# Autodesk Inventor assembly: J005687
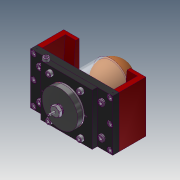
[picture p0: Inventor's stored thumbnail of the model, 180x180]
Saved by Autodesk Inventor 2015 SP1 (Build 190203100, 203)
## iProperties
Created: 2010-04-29
Part Number: J005687
Document SubType Name: Assembly
Designer: InventorUser
Description: CANNON AND HOLDER ASSY
Vendor: HHMI: JRC - ID&F
ALTERED ITEM DESCRIPTION: N/A
DESIGN DEPARTMENT: HHMI: JRC - ID&F
Revision Number: 0
## Documents named in this file (11)
- C:\_WORKSPACE\DATA\COLLABORATION\SVOBODA LAB\MOUSE POSITIONING SYSTEMS\MCAD\BALL SETUP\MBS AssemblyCanHolder.iam
- C:\_WORKSPACE\DATA\COLLABORATION\SVOBODA LAB\MOUSE POSITIONING SYSTEMS\MCAD\BALL SETUP\Ball_Rig\CanClamp.ipt
- C:\_WORKSPACE\DATA\COLLABORATION\SVOBODA LAB\MOUSE POSITIONING SYSTEMS\MCAD\BALL SETUP\Ball_Rig\CanClamper16.ipt
- C:\_WORKSPACE\DATA\COLLABORATION\SVOBODA LAB\MOUSE POSITIONING SYSTEMS\MCAD\BALL SETUP\Ball_Rig\ClamperPlate.ipt
- C:\_WORKSPACE\DATA\COLLABORATION\SVOBODA LAB\MOUSE POSITIONING SYSTEMS\MCAD\BALL SETUP\Ball_Rig\PingPongBall.ipt
- C:\_WORKSPACE\DATA\COLLABORATION\SVOBODA LAB\MOUSE POSITIONING SYSTEMS\MCAD\BALL SETUP\50745K150.ipt
- C:\_WORKSPACE\DATA\COLLABORATION\SVOBODA LAB\MOUSE POSITIONING SYSTEMS\MCAD\BALL SETUP\92185A203.ipt
- C:\_WORKSPACE\DATA\COLLABORATION\SVOBODA LAB\MOUSE POSITIONING SYSTEMS\MCAD\BALL SETUP\92185A194.ipt
- C:\_WORKSPACE\DATA\COLLABORATION\SVOBODA LAB\MOUSE POSITIONING SYSTEMS\MCAD\BALL SETUP\90291A578.ipt
- C:\_WORKSPACE\DATA\COLLABORATION\SVOBODA LAB\MOUSE POSITIONING SYSTEMS\MCAD\BALL SETUP\Ball_Rig\BottomCapAirBall.ipt
- C:\_WORKSPACE\DATA\COLLABORATION\SVOBODA LAB\MOUSE POSITIONING SYSTEMS\MCAD\BALL SETUP\Ball_Rig\BallHolderTubeAirBall.ipt
## Components (23 placed, 10 different names)
1. CanClamp:1 — Mate:1, Mate:2, Mate:7, Mate:8, Mate:12, Mate:13, Mate:34, Mate:35, Mate:36, Mate:37, Mate:38, Mate:39, Mate:40, Mate:41
2. CanClamper16:1 — Mate:3, Mate:4
3. CanClamper16:2 — Mate:5, Mate:6
4. ClamperPlate:1 — Mate:1, Mate:2, Mate:3, Mate:4, Mate:5, Mate:6, Mate:7, Mate:8, Mate:14, Mate:15, Mate:16, Mate:17, Mate:18, Mate:19, Mate:20, Mate:21, Mate:22, Mate:23, Mate:24, Mate:25, Mate:26, Mate:27, Flush:1, Mate:28, Flush:2, Mate:29, Flush:3, Mate:30, Flush:4
5. PingPongBall:1
6. 50745K150:1
7. 92185A203:1 — Mate:12, Mate:13
8. 92185A194:1 — Mate:14, Mate:15
9. 92185A194:2 — Mate:16, Mate:17
10. 92185A194:3 — Mate:18, Mate:19, Mate:20
11. 92185A194:4 — Mate:25, Mate:26
12. 92185A194:5 — Mate:23, Mate:24
13. 92185A194:6 — Mate:21, Mate:22
14. 90291A578:1 — Mate:28, Flush:2
15. 90291A578:2 — Mate:27, Flush:1
16. 90291A578:3 — Mate:29, Flush:3
17. 90291A578:4 — Mate:30, Flush:4
18. BottomCapAirBall:1
19. BallHolderTubeAirBall:1
20. 92185A194:7 — Mate:34, Mate:35
21. 92185A194:8 — Mate:36, Mate:37
22. 92185A194:9 — Mate:40, Mate:41
23. 92185A194:10 — Mate:38, Mate:39
## Relationships (46: Mate 41, Flush 4, Insert 1)
- Mate:1: CanClamp:1 ↔ ClamperPlate:1
- Mate:2: CanClamp:1 ↔ ClamperPlate:1
- Mate:3: CanClamper16:1 ↔ ClamperPlate:1
- Mate:4: CanClamper16:1 ↔ ClamperPlate:1
- Mate:5: CanClamper16:2 ↔ ClamperPlate:1
- Mate:6: CanClamper16:2 ↔ ClamperPlate:1
- Mate:7: CanClamp:1 ↔ ClamperPlate:1
- Mate:8: CanClamp:1 ↔ ClamperPlate:1
- [Insert] (-1.905 mm): CanClamp:1 ↔ BallHolderTubeAirBall:1
- [Mate]: PingPongBall:1 ↔ BallHolderTubeAirBall:1
- [Mate]: 50745K150:1 ↔ BottomCapAirBall:1
- [Mate] (2.54 mm): 50745K150:1 ↔ BottomCapAirBall:1
- Mate:12: CanClamp:1 ↔ 92185A203:1
- Mate:13: CanClamp:1 ↔ 92185A203:1
- Mate:14: ClamperPlate:1 ↔ 92185A194:1
- Mate:15: ClamperPlate:1 ↔ 92185A194:1
- Mate:16: ClamperPlate:1 ↔ 92185A194:2
- Mate:17: ClamperPlate:1 ↔ 92185A194:2
- Mate:18: ClamperPlate:1 ↔ 92185A194:3
- Mate:19: ClamperPlate:1 ↔ 92185A194:3
- Mate:20: ClamperPlate:1 ↔ 92185A194:3
- Mate:21: ClamperPlate:1 ↔ 92185A194:6
- Mate:22: ClamperPlate:1 ↔ 92185A194:6
- Mate:23: ClamperPlate:1 ↔ 92185A194:5
- Mate:24: ClamperPlate:1 ↔ 92185A194:5
- Mate:25: ClamperPlate:1 ↔ 92185A194:4
- Mate:26: ClamperPlate:1 ↔ 92185A194:4
- Mate:27: ClamperPlate:1 ↔ 90291A578:2
- Flush:1 (-2.54 mm): ClamperPlate:1 ↔ 90291A578:2
- Mate:28: ClamperPlate:1 ↔ 90291A578:1
- Flush:2 (-2.54 mm): ClamperPlate:1 ↔ 90291A578:1
- Mate:29: ClamperPlate:1 ↔ 90291A578:3
- Flush:3 (-2.54 mm): ClamperPlate:1 ↔ 90291A578:3
- Mate:30: ClamperPlate:1 ↔ 90291A578:4
- Flush:4 (-2.54 mm): ClamperPlate:1 ↔ 90291A578:4
- [Mate]: BottomCapAirBall:1 ↔ BallHolderTubeAirBall:1
- [Mate]: BottomCapAirBall:1 ↔ BallHolderTubeAirBall:1
- [Mate]: BottomCapAirBall:1 ↔ BallHolderTubeAirBall:1
- Mate:34: CanClamp:1 ↔ 92185A194:7
- Mate:35: CanClamp:1 ↔ 92185A194:7
- Mate:36: CanClamp:1 ↔ 92185A194:8
- Mate:37: CanClamp:1 ↔ 92185A194:8
- Mate:38: CanClamp:1 ↔ 92185A194:10
- Mate:39: CanClamp:1 ↔ 92185A194:10
- Mate:40: CanClamp:1 ↔ 92185A194:9
- Mate:41: CanClamp:1 ↔ 92185A194:9
## Named parameters: d53_d0 = 0 mm, d54_d1 = 0 mm, d55_d2 = 0 mm
